# Autodesk Inventor assembly: Montagem_case
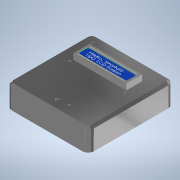
[picture p0: Inventor's stored thumbnail of the model, 180x180]
Saved by Autodesk Inventor 2021 (Build 250183000, 183)
## iProperties
Created: 2020-12-21
Part Number: Montagem_case
Document SubType Name: Assembly
Designer: Vitor
Author: Vitor
## iProperties of the stored document 402530, LiPo battery 300 mAh.ipt
Created: 2017-02-28
Part Number: 402530, LiPo battery 300 mAh
Material: Generic
Document SubType Name: Modeling
Designer: Vitor
Density: 1 g/cm^3
Appearance: Default
Author: Vitor
Sending System: SolidWorks 2016
Last Author: sbastiani
Last Saved: 2017-04-03
## iProperties of the stored document LCD Screen.ipt
Created: 2020-09-17
Part Number: LCD Screen
Material: Generic
Description: STEP AP214
Document SubType Name: Modeling
Designer: Vitor
Density: 1 g/cm^3
Appearance: Default
Title: LCD Screen.STEP
Revision Number: ANY
Sending System: SolidWorks 2018
Preprocessor: SwSTEP 2.0
## Documents named in this file (8)
- **C:\Users\Vitor\Desktop\Projeto Sensor de sal - LaisUFRN\3d_models\Case\Montagem_case.iam*LocalDocs*xAaaaq5aaAaaaaaaaAaaaayj51b*402530, LiPo battery 300 mAh.ipt
- **C:\Users\Vitor\Desktop\Projeto Sensor de sal - LaisUFRN\3d_models\Case\Montagem_case.iam*LocalDocs*xAaaaqdbaAaaaaaaaAaaaqyb2Ug*LCD Screen.ipt
- C:\Users\Vitor\Desktop\Projeto Sensor de sal - LaisUFRN\3d_models\Case\Montagem_case.iam
- C:\Users\Vitor\Desktop\Projeto Sensor de sal - LaisUFRN\3d_models\Case\Base.ipt
- C:\Users\Vitor\Desktop\Projeto Sensor de sal - LaisUFRN\3d_models\PCB\Inventor_files\esquematico.iam
- C:\Users\Vitor\Desktop\Projeto Sensor de sal - LaisUFRN\3d_models\Case\Tampa.ipt
- C:\Users\Vitor\Desktop\Projeto Sensor de sal - LaisUFRN\3d_models\Case\LCD Screen.STEP
- C:\Users\Vitor\Desktop\Projeto Sensor de sal - LaisUFRN\3d_models\Case\402530, LiPo battery 300 mAh.SLDPRT
## Components (5 placed, 5 different names)
1. Base:1 — Mate:1, Mate:2, Mate:3, Mate:4, Mate:8
2. esquematico:1 [sub-assembly] — Mate:1, Mate:2
3. Tampa:1 — Mate:3, Mate:4, Mate:5, Mate:6, Mate:7
4. LCD Screen:1 — Mate:5, Mate:6, Mate:7
5. 402530, LiPo battery 300 mAh:1 — Mate:8
## Relationships (8: Mate 8)
- Mate:1: Base:1 ↔ esquematico:1
- Mate:2: Base:1 ↔ esquematico:1
- Mate:3: Base:1 ↔ Tampa:1
- Mate:4: Base:1 ↔ Tampa:1
- Mate:5: Tampa:1 ↔ LCD Screen:1
- Mate:6: Tampa:1 ↔ LCD Screen:1
- Mate:7: Tampa:1 ↔ LCD Screen:1
- Mate:8: Base:1 ↔ 402530, LiPo battery 300 mAh:1
